# Autodesk Inventor assembly: Assembly1
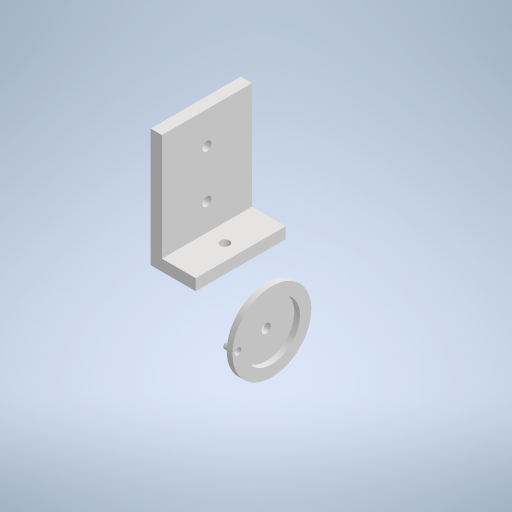
[picture p0: Inventor's stored thumbnail of the model, 512x512]
Saved by Autodesk Inventor 2024 (Build 280153000, 153)
## iProperties
Created: 2024-02-08
Part Number: Assembly1
Document SubType Name: Assembly
Designer: haris
Author: haris
## Documents named in this file (3)
- C:\Users\haris\OneDrive\Desktop\Assembly1.iam
- C:\Users\haris\OneDrive\Desktop\Support_plate.ipt
- C:\Users\haris\OneDrive\Desktop\Geneva_driver.ipt
## Components (2 placed, 2 different names)
1. Support_plate:1 — Mate:1, Mate:2, Mate:3, Mate:4
2. Geneva_driver:1 — Mate:1, Mate:2, Mate:3, Mate:4
## Relationships (4: Mate 4)
- Mate:1: Support_plate:1 ↔ Geneva_driver:1
- Mate:2: Support_plate:1 ↔ Geneva_driver:1
- Mate:3: Support_plate:1 ↔ Geneva_driver:1
- Mate:4: Support_plate:1 ↔ Geneva_driver:1
